# Autodesk Inventor assembly: nakladkacomplete
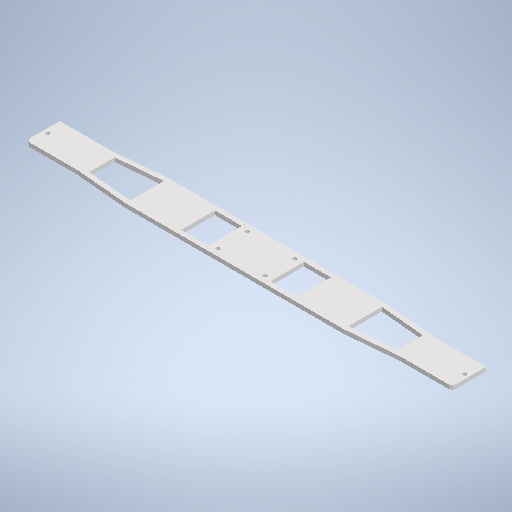
[picture p0: Inventor's stored thumbnail of the model, 512x512]
Saved by Autodesk Inventor 2025.3 (Build 293356000, 356)
## iProperties
Created: 2026-04-21
Part Number: nakladkacomplete
Document SubType Name: Assembly
Designer: ksawe
Author: ksawe
## Documents named in this file (2)
- C:\Users\ksawe\OneDrive\Pulpit\Exomy v1\wersja3\nakladkacomplete.iam
- C:\Users\ksawe\OneDrive\Pulpit\Exomy v1\wersja3\nakladkapart1.ipt
## Components (2 placed, 1 different names)
1. nakladkapart1:1 — Mate:1, Mate:2, Mate:3
2. nakladkapart1:2 — Mate:1, Mate:2, Mate:3
## Relationships (3: Mate 3)
- Mate:1: nakladkapart1:1 ↔ nakladkapart1:2
- Mate:2: nakladkapart1:1 ↔ nakladkapart1:2
- Mate:3: nakladkapart1:1 ↔ nakladkapart1:2
